# Autodesk Inventor assembly: Sternum Assembly
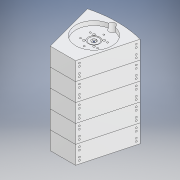
[picture p0: Inventor's stored thumbnail of the model, 180x180]
Saved by Autodesk Inventor 2017 SP1 (Build 210196100, 196)
## iProperties
Created: 2017-09-17
Part Number: Sternum Assembly
Document SubType Name: Assembly
Designer: Zach
Author: Zach
## Documents named in this file (7)
- C:\Users\Zach\Documents\GitHub\tr1\src\Body\Chest Assembly\Sternum Assembly\Sternum Assembly.iam
- C:\Users\Zach\Documents\GitHub\tr1\src\Body\Chest Assembly\Sternum Assembly\SA001.ipt
- C:\Users\Zach\Documents\GitHub\tr1\src\Body\Chest Assembly\Sternum Assembly\SA002.ipt
- C:\Users\Zach\Documents\GitHub\tr1\src\Body\Chest Assembly\Sternum Assembly\SA004.ipt
- C:\Users\Zach\Documents\GitHub\tr1\lib\Stepper Motor - NEMA 17\NEMA17.ipt
- C:\Users\Zach\Documents\GitHub\tr1\src\Body\Chest Assembly\Sternum Assembly\SA003.ipt
- C:\Users\Zach\Documents\GitHub\tr1\src\Body\Chest Assembly\Sternum Assembly\SA005.ipt
## Components (7 placed, 6 different names)
1. SA001:1 — Mate:1, Mate:2, Mate:3, Mate:4, Mate:11, Mate:12, Mate:13, Mate:23
2. SA002:1 — Mate:5, Mate:10, Mate:11, Mate:12, Mate:13, Mate:14, Mate:15, Mate:16, Mate:17
3. SA004:1 — Mate:5, Mate:6, Mate:7
4. NEMA17:1 — Mate:6, Mate:7, Mate:10, Mate:14
5. SA003:1 — Mate:15, Mate:16, Mate:17, Mate:18, Mate:19, Mate:20
6. SA005:1 — Mate:18, Mate:19, Mate:20, Mate:21, Mate:22
7. SA005:2 — Mate:21, Mate:22, Mate:23
## Relationships (21: Mate 21)
- Mate:1: SA001:1
- Mate:2: SA001:1
- Mate:3: SA001:1
- Mate:4: SA001:1
- Mate:5: SA002:1 ↔ SA004:1
- Mate:6: SA004:1 ↔ NEMA17:1
- Mate:7: SA004:1 ↔ NEMA17:1
- Mate:10: SA002:1 ↔ NEMA17:1
- Mate:11: SA001:1 ↔ SA002:1
- Mate:12: SA001:1 ↔ SA002:1
- Mate:13: SA001:1 ↔ SA002:1
- Mate:14: SA002:1 ↔ NEMA17:1
- Mate:15: SA002:1 ↔ SA003:1
- Mate:16: SA002:1 ↔ SA003:1
- Mate:17: SA002:1 ↔ SA003:1
- Mate:18: SA003:1 ↔ SA005:1
- Mate:19: SA003:1 ↔ SA005:1
- Mate:20: SA003:1 ↔ SA005:1
- Mate:21: SA005:1 ↔ SA005:2
- Mate:22: SA005:1 ↔ SA005:2
- Mate:23: SA001:1 ↔ SA005:2
